# Autodesk Inventor assembly: teljes3
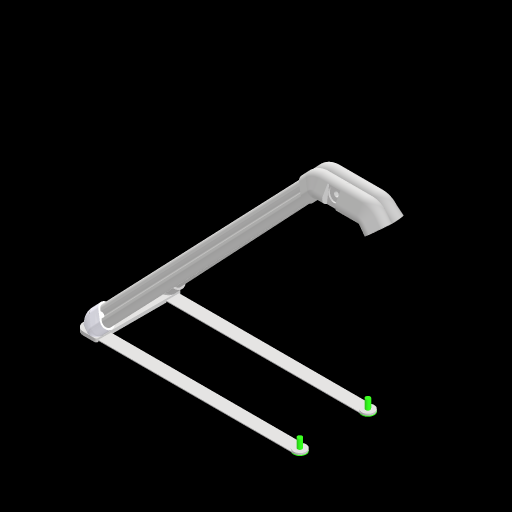
[picture p0: Inventor's stored thumbnail of the model, 512x512]
Saved by Autodesk Inventor 2023 (Build 270158000, 158)
## iProperties
Created: 2022-11-11
Part Number: teljes3
Document SubType Name: Assembly
Designer: gd1
Author: gd1
## Documents named in this file (7)
- C:\Users\gd1\3D Objects\3D nagyteherbírású híd\Híd\H-d\teljes3.iam
- C:\Users\gd1\3D Objects\3D nagyteherbírású híd\Híd\H-d\45 fok középre.ipt
- C:\Users\gd1\3D Objects\3D nagyteherbírású híd\Híd\H-d\palca 325mm.ipt
- C:\Users\gd1\3D Objects\3D nagyteherbírású híd\Híd\H-d\kozepso szalag2.ipt
- C:\Users\gd1\3D Objects\3D nagyteherbírású híd\Híd\H-d\45 fok kozepcsati.ipt.iam
- C:\Users\gd1\3D Objects\3D nagyteherbírású híd\Híd\H-d\tipli.ipt
- 45 fok kozepcsati.ipt
## Components (10 placed, 5 different names)
1. 45 fok középre:1 — Rotational:1, Rotational:2, Rotational:7, Rotational:8
2. palca 325mm:1 — Rotational:2
3. palca 325mm:2 — Rotational:1
4. 45 fok kozepcsati.ipt:1 [sub-assembly]
5. kozepso szalag2:1 — Rotational:7, Rotational:9, Rotational:11
6. kozepso szalag2:2 — Rotational:8, Rotational:10, Rotational:12
7. tipli:1 — Rotational:9
8. tipli:2 — Rotational:10
9. tipli:3 — Rotational:11
10. tipli:4 — Rotational:12
## Relationships (8: RevoluteJoint 8)
- Rotational:1 [RevoluteJoint]: 45 fok középre:1 ↔ palca 325mm:2
- Rotational:2 [RevoluteJoint]: 45 fok középre:1 ↔ palca 325mm:1
- Rotational:7 [RevoluteJoint]: 45 fok középre:1 ↔ kozepso szalag2:1
- Rotational:8 [RevoluteJoint]: 45 fok középre:1 ↔ kozepso szalag2:2
- Rotational:9 [RevoluteJoint]: kozepso szalag2:1 ↔ tipli:1
- Rotational:10 [RevoluteJoint]: kozepso szalag2:2 ↔ tipli:2
- Rotational:11 [RevoluteJoint]: kozepso szalag2:1 ↔ tipli:3
- Rotational:12 [RevoluteJoint]: kozepso szalag2:2 ↔ tipli:4
